# Autodesk Inventor assembly: 000-belt_liner_v5
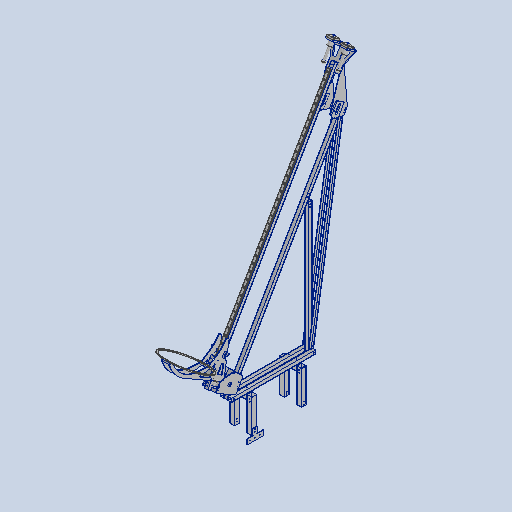
[picture p0: Inventor's stored thumbnail of the model, 512x512]
Saved by Autodesk Inventor 2025.2 (Build 292293000, 293)
## iProperties
Created: 2025-02-22
Part Number: 000-belt_liner_v5
Document SubType Name: Assembly
Designer: haruy
Author: haruy
## Documents named in this file (22)
- C:\Users\haruy\Documents\ロボコン\NHK2025\cad\nagahisa\belt_liner\000-belt_liner_v5.iam
- C:\Users\haruy\Documents\ロボコン\NHK2025\cad\nagahisa\belt_liner\belt_liner_v5_ASP_Base.ipt
- C:\Users\haruy\Documents\ロボコン\NHK2025\cad\nagahisa\belt_liner\SSE2B-MX13-970.iam
- C:\Users\haruy\Documents\ロボコン\NHK2025\cad\nagahisa\belt_liner\belt_liner_v5_Plate_1.ipt
- C:\Users\haruy\Documents\ロボコン\NHK2025\cad\nagahisa\belt_liner\belt_liner_v5_Plate_2.ipt
- C:\Users\haruy\Documents\ロボコン\NHK2025\cad\nagahisa\belt_liner\belt_liner_v5_Plate_3.ipt
- C:\Users\haruy\Documents\ロボコン\NHK2025\cad\nagahisa\belt_liner\belt_liner_v5_Plate_4.ipt
- C:\Users\haruy\Documents\ロボコン\NHK2025\cad\nagahisa\belt_liner\belt_liner_v5_Plate_5.ipt
- C:\Users\haruy\Documents\ロボコン\NHK2025\cad\nagahisa\belt_liner\belt_liner_v5_Plate_6.ipt
- C:\Users\haruy\Documents\ロボコン\NHK2025\cad\nagahisa\belt_liner\belt_liner_v1_Plate_9.ipt
- C:\Users\haruy\Documents\ロボコン\NHK2025\cad\nagahisa\belt_liner\belt_liner_v5_Plate_7.ipt
- C:\Users\haruy\Documents\ロボコン\NHK2025\cad\nagahisa\belt_liner\belt_liner_v5_Plate_8.ipt
- C:\Users\haruy\Documents\ロボコン\NHK2025\cad\nagahisa\belt_liner\belt_liner_v5_Plate_9.ipt
- C:\Users\haruy\Documents\ロボコン\NHK2025\cad\nagahisa\belt_liner\belt_liner_v2_Pom_r.ipt
- C:\Users\haruy\Documents\ロボコン\NHK2025\cad\nagahisa\belt_liner\belt_liner_v5_Plate_10.ipt
- C:\Users\haruy\Documents\ロボコン\NHK2025\cad\nagahisa\belt_liner\belt_liner_v5_shaft_1.ipt
- C:\Users\haruy\Documents\ロボコン\NHK2025\cad\nagahisa\belt_liner\gomu_leg.ipt
- C:\Users\haruy\Documents\ロボコン\NHK2025\cad\nagahisa\belt_liner\belt_liner_v5_Plate_11.ipt
- C:\Users\haruy\Documents\ロボコン\NHK2025\cad\nagahisa\belt_liner\belt_liner_v5_Plate_12.ipt
- C:\Users\haruy\Documents\ロボコン\NHK2025\cad\nagahisa\belt_liner\C-LHFS10.ipt
- C:\Users\haruy\Documents\ロボコン\NHK2025\cad\nagahisa\belt_liner\belt_liner_v5_shaft_2.ipt
- C:\Users\haruy\Documents\ロボコン\NHK2025\cad\nagahisa\belt_liner\belt_liner_v5_Plate_13.ipt
## Components (35 placed, 21 different names)
1. belt_liner_v5_ASP_Base:1 — 挿入:1, 挿入:2, 挿入:3, 挿入:4, 挿入:5, 挿入:6, 挿入:11, 挿入:12, 挿入:15, 挿入:16, 挿入:17, 挿入:18, 挿入:62, 挿入:63
2. SSE2B-MX13-970:1 [sub-assembly] — 挿入:1, 挿入:2, 挿入:3, 挿入:4, 挿入:28, 挿入:29
3. belt_liner_v5_Plate_1:1 — 挿入:7, 挿入:8, 挿入:13, 挿入:14
4. belt_liner_v5_Plate_2:1 — 挿入:5, 挿入:6, 挿入:7, 挿入:8, 挿入:9, 挿入:10, 挿入:38, 挿入:39, 挿入:40, 挿入:41
5. belt_liner_v5_Plate_1:2 — 挿入:9, 挿入:10
6. belt_liner_v5_Plate_3:1 — 挿入:11, 挿入:12, 挿入:13, 挿入:14
7. belt_liner_v5_Plate_4:1 — 挿入:15, 挿入:16
8. belt_liner_v5_Plate_5:1 — 挿入:17, 挿入:18, 挿入:19, 挿入:20, 挿入:21, 挿入:22, 挿入:54, 挿入:55, 挿入:56, 挿入:57
9. belt_liner_v5_Plate_6:1 — 挿入:19, 挿入:20, 挿入:23, 挿入:24, 挿入:25
10. belt_liner_v5_Plate_6:2 — 挿入:21, 挿入:22, 挿入:26, 挿入:27
11. belt_liner_v1_Plate_9:1 — 挿入:23, 挿入:24, 挿入:25
12. belt_liner_v1_Plate_9:2 — 挿入:26, 挿入:27
13. belt_liner_v5_Plate_7:1 — 挿入:30, 挿入:31, 挿入:34, 挿入:35, フラッシュ:1, フラッシュ:2, 挿入:46, 挿入:47
14. belt_liner_v5_Plate_8:1 — 挿入:28, 挿入:29, 挿入:30, 挿入:31, 挿入:32, 挿入:33
15. belt_liner_v5_Plate_7:2 — 挿入:32, 挿入:33, 挿入:48, 挿入:49
16. belt_liner_v5_Plate_9:1 — 挿入:34, フラッシュ:2, 挿入:37
17. belt_liner_v5_Plate_9:2 — 挿入:35, フラッシュ:1, 挿入:36
18. belt_liner_v2_Pom_r:1 — 挿入:36, 挿入:37
19. belt_liner_v5_Plate_10:1 — 挿入:40, 挿入:41, 挿入:43
20. belt_liner_v5_Plate_10:2 — 挿入:38, 挿入:39, 挿入:42
21. belt_liner_v5_shaft_1:1 — 挿入:42, 挿入:44
22. belt_liner_v5_shaft_1:2 — 挿入:43, 挿入:45
23. gomu_leg:1 — 挿入:45
24. gomu_leg:2 — 挿入:44
25. belt_liner_v5_Plate_11:1 — 挿入:46, 挿入:47
26. belt_liner_v5_Plate_11:2 — 挿入:48, 挿入:49
27. belt_liner_v5_Plate_12:1 — 挿入:52, 挿入:53, 挿入:54, 挿入:55
28. C-LHFS10:1 — 挿入:52, 挿入:53, 挿入:58
29. belt_liner_v5_Plate_12:2 — 挿入:50, 挿入:51, 挿入:56, 挿入:57
30. C-LHFS10:2 — 挿入:50, 挿入:51, 挿入:59
31. belt_liner_v5_shaft_2:1 — 挿入:59, 挿入:61
32. belt_liner_v5_shaft_2:2 — 挿入:58, 挿入:60
33. gomu_leg:3 — 挿入:61
34. gomu_leg:4 — 挿入:60
35. belt_liner_v5_Plate_13:1 — 挿入:62, 挿入:63
## Relationships (65: Insert 63, Flush 2)
- 挿入:1 [Insert]: belt_liner_v5_ASP_Base:1 ↔ SSE2B-MX13-970:1
- 挿入:2 [Insert]: belt_liner_v5_ASP_Base:1 ↔ SSE2B-MX13-970:1
- 挿入:3 [Insert]: belt_liner_v5_ASP_Base:1 ↔ SSE2B-MX13-970:1
- 挿入:4 [Insert]: belt_liner_v5_ASP_Base:1 ↔ SSE2B-MX13-970:1
- 挿入:5 [Insert]: belt_liner_v5_ASP_Base:1 ↔ belt_liner_v5_Plate_2:1
- 挿入:6 [Insert]: belt_liner_v5_ASP_Base:1 ↔ belt_liner_v5_Plate_2:1
- 挿入:7 [Insert]: belt_liner_v5_Plate_1:1 ↔ belt_liner_v5_Plate_2:1
- 挿入:8 [Insert]: belt_liner_v5_Plate_1:1 ↔ belt_liner_v5_Plate_2:1
- 挿入:9 [Insert]: belt_liner_v5_Plate_2:1 ↔ belt_liner_v5_Plate_1:2
- 挿入:10 [Insert]: belt_liner_v5_Plate_2:1 ↔ belt_liner_v5_Plate_1:2
- 挿入:11 [Insert]: belt_liner_v5_ASP_Base:1 ↔ belt_liner_v5_Plate_3:1
- 挿入:12 [Insert]: belt_liner_v5_ASP_Base:1 ↔ belt_liner_v5_Plate_3:1
- 挿入:13 [Insert]: belt_liner_v5_Plate_1:1 ↔ belt_liner_v5_Plate_3:1
- 挿入:14 [Insert]: belt_liner_v5_Plate_1:1 ↔ belt_liner_v5_Plate_3:1
- 挿入:15 [Insert]: belt_liner_v5_ASP_Base:1 ↔ belt_liner_v5_Plate_4:1
- 挿入:16 [Insert]: belt_liner_v5_ASP_Base:1 ↔ belt_liner_v5_Plate_4:1
- 挿入:17 [Insert]: belt_liner_v5_ASP_Base:1 ↔ belt_liner_v5_Plate_5:1
- 挿入:18 [Insert]: belt_liner_v5_ASP_Base:1 ↔ belt_liner_v5_Plate_5:1
- 挿入:19 [Insert]: belt_liner_v5_Plate_5:1 ↔ belt_liner_v5_Plate_6:1
- 挿入:20 [Insert]: belt_liner_v5_Plate_5:1 ↔ belt_liner_v5_Plate_6:1
- 挿入:21 [Insert]: belt_liner_v5_Plate_5:1 ↔ belt_liner_v5_Plate_6:2
- 挿入:22 [Insert]: belt_liner_v5_Plate_5:1 ↔ belt_liner_v5_Plate_6:2
- 挿入:23 [Insert]: belt_liner_v5_Plate_6:1 ↔ belt_liner_v1_Plate_9:1
- 挿入:24 [Insert]: belt_liner_v5_Plate_6:1 ↔ belt_liner_v1_Plate_9:1
- 挿入:25 [Insert]: belt_liner_v5_Plate_6:1 ↔ belt_liner_v1_Plate_9:1
- 挿入:26 [Insert]: belt_liner_v5_Plate_6:2 ↔ belt_liner_v1_Plate_9:2
- 挿入:27 [Insert]: belt_liner_v5_Plate_6:2 ↔ belt_liner_v1_Plate_9:2
- 挿入:28 [Insert]: SSE2B-MX13-970:1 ↔ belt_liner_v5_Plate_8:1
- 挿入:29 [Insert]: SSE2B-MX13-970:1 ↔ belt_liner_v5_Plate_8:1
- 挿入:30 [Insert]: belt_liner_v5_Plate_7:1 ↔ belt_liner_v5_Plate_8:1
- 挿入:31 [Insert]: belt_liner_v5_Plate_7:1 ↔ belt_liner_v5_Plate_8:1
- 挿入:32 [Insert]: belt_liner_v5_Plate_8:1 ↔ belt_liner_v5_Plate_7:2
- 挿入:33 [Insert]: belt_liner_v5_Plate_8:1 ↔ belt_liner_v5_Plate_7:2
- 挿入:34 [Insert]: belt_liner_v5_Plate_7:1 ↔ belt_liner_v5_Plate_9:1
- 挿入:35 [Insert]: belt_liner_v5_Plate_7:1 ↔ belt_liner_v5_Plate_9:2
- フラッシュ:1 [Flush]: belt_liner_v5_Plate_7:1 ↔ belt_liner_v5_Plate_9:2
- フラッシュ:2 [Flush]: belt_liner_v5_Plate_7:1 ↔ belt_liner_v5_Plate_9:1
- 挿入:36 [Insert]: belt_liner_v5_Plate_9:2 ↔ belt_liner_v2_Pom_r:1
- 挿入:37 [Insert]: belt_liner_v5_Plate_9:1 ↔ belt_liner_v2_Pom_r:1
- 挿入:38 [Insert]: belt_liner_v5_Plate_2:1 ↔ belt_liner_v5_Plate_10:2
- 挿入:39 [Insert]: belt_liner_v5_Plate_2:1 ↔ belt_liner_v5_Plate_10:2
- 挿入:40 [Insert]: belt_liner_v5_Plate_2:1 ↔ belt_liner_v5_Plate_10:1
- 挿入:41 [Insert]: belt_liner_v5_Plate_2:1 ↔ belt_liner_v5_Plate_10:1
- 挿入:42 [Insert]: belt_liner_v5_Plate_10:2 ↔ belt_liner_v5_shaft_1:1
- 挿入:43 [Insert]: belt_liner_v5_Plate_10:1 ↔ belt_liner_v5_shaft_1:2
- 挿入:44 [Insert]: belt_liner_v5_shaft_1:1 ↔ gomu_leg:2
- 挿入:45 [Insert]: belt_liner_v5_shaft_1:2 ↔ gomu_leg:1
- 挿入:46 [Insert]: belt_liner_v5_Plate_7:1 ↔ belt_liner_v5_Plate_11:1
- 挿入:47 [Insert]: belt_liner_v5_Plate_7:1 ↔ belt_liner_v5_Plate_11:1
- 挿入:48 [Insert]: belt_liner_v5_Plate_7:2 ↔ belt_liner_v5_Plate_11:2
- 挿入:49 [Insert]: belt_liner_v5_Plate_7:2 ↔ belt_liner_v5_Plate_11:2
- 挿入:50 [Insert]: belt_liner_v5_Plate_12:2 ↔ C-LHFS10:2
- 挿入:51 [Insert]: belt_liner_v5_Plate_12:2 ↔ C-LHFS10:2
- 挿入:52 [Insert]: belt_liner_v5_Plate_12:1 ↔ C-LHFS10:1
- 挿入:53 [Insert]: belt_liner_v5_Plate_12:1 ↔ C-LHFS10:1
- 挿入:54 [Insert]: belt_liner_v5_Plate_5:1 ↔ belt_liner_v5_Plate_12:1
- 挿入:55 [Insert]: belt_liner_v5_Plate_5:1 ↔ belt_liner_v5_Plate_12:1
- 挿入:56 [Insert]: belt_liner_v5_Plate_5:1 ↔ belt_liner_v5_Plate_12:2
- 挿入:57 [Insert]: belt_liner_v5_Plate_5:1 ↔ belt_liner_v5_Plate_12:2
- 挿入:58 [Insert] (-34 mm): C-LHFS10:1 ↔ belt_liner_v5_shaft_2:2
- 挿入:59 [Insert] (-34 mm): C-LHFS10:2 ↔ belt_liner_v5_shaft_2:1
- 挿入:60 [Insert]: belt_liner_v5_shaft_2:2 ↔ gomu_leg:4
- 挿入:61 [Insert]: belt_liner_v5_shaft_2:1 ↔ gomu_leg:3
- 挿入:62 [Insert]: belt_liner_v5_ASP_Base:1 ↔ belt_liner_v5_Plate_13:1
- 挿入:63 [Insert]: belt_liner_v5_ASP_Base:1 ↔ belt_liner_v5_Plate_13:1
